# Autodesk Inventor assembly: SMC MSQ Rotary Pneumatic Rack and Pinion Rotary Table Block
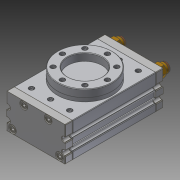
[picture p0: Inventor's stored thumbnail of the model, 180x180]
Saved by Autodesk Inventor 2014 SP1 (Build 180222100, 222)
## iProperties
Created: 2013-12-16
Part Number: SMC MSQ Rotary Pneumatic Rack and Pinion Rotary Table Block
Document SubType Name: Assembly
Designer: Moses
Mass: 511.529 g
Surface Area: 776.899 cm^2
Volume: 450.572 cm^3
Density: 1.13529 g/cm^3
Author: Moses
## Documents named in this file (7)
- C:\Users\Moses\Documents\Inventor\Sally Rebuild\Rebuild Sally\SMC MSQ Rotary Pneumatic Rack and Pinion Rotary Table Block.iam
- C:\Users\Moses\Documents\Inventor\Sally Rebuild\Rebuild Sally\Rotary Pneumatic Cylinder Body.ipt
- C:\Users\Moses\Documents\Inventor\Sally Rebuild\Rebuild Sally\Rotary Pneumatic Cylinder Front End.ipt
- C:\Users\Moses\Documents\Inventor\Sally Rebuild\Rebuild Sally\Rotary Pneumatic Cylinder Back End.ipt
- C:\Users\Moses\Documents\Inventor\Sally Rebuild\Rebuild Sally\Rotary Pneumatic Cylinder Axis.ipt
- C:\Users\Moses\Documents\Inventor\Sally Rebuild\Rebuild Sally\Pneumatics\Pneumatics_SMC_KQ2H07-35S.ipt
- C:\Users\Moses\Documents\Inventor\Sally Rebuild\Rebuild Sally\10-32x0625_shcs.ipt
## Components (14 placed, 6 different names)
1. Rotary Pneumatic Cylinder Body:1 — Mate:1, Flush:1, Flush:2, Mate:2, Flush:3, Flush:4, Insert:1
2. Rotary Pneumatic Cylinder Front End:1 — Mate:1, Flush:1, Flush:2, Insert:8, Insert:9, Insert:10, Insert:11
3. Rotary Pneumatic Cylinder Back End:1 — Mate:2, Flush:3, Flush:4, Insert:2, Insert:3, Insert:4, Insert:5, Insert:6, Insert:7
4. Rotary Pneumatic Cylinder Axis:1 — Insert:1
5. Pneumatics_SMC_KQ2H07-35S:1 — Insert:2
6. Pneumatics_SMC_KQ2H07-35S:2 — Insert:3
7. 10-32x0625_shcs:1 — Insert:4
8. 10-32x0625_shcs:2 — Insert:5
9. 10-32x0625_shcs:3 — Insert:6
10. 10-32x0625_shcs:4 — Insert:7
11. 10-32x0625_shcs:5 — Insert:8
12. 10-32x0625_shcs:6 — Insert:9
13. 10-32x0625_shcs:7 — Insert:10
14. 10-32x0625_shcs:8 — Insert:11
## Relationships (17: Insert 11, Flush 4, Mate 2)
- Mate:1: Rotary Pneumatic Cylinder Body:1 ↔ Rotary Pneumatic Cylinder Front End:1
- Flush:1: Rotary Pneumatic Cylinder Body:1 ↔ Rotary Pneumatic Cylinder Front End:1
- Flush:2: Rotary Pneumatic Cylinder Body:1 ↔ Rotary Pneumatic Cylinder Front End:1
- Mate:2: Rotary Pneumatic Cylinder Body:1 ↔ Rotary Pneumatic Cylinder Back End:1
- Flush:3: Rotary Pneumatic Cylinder Body:1 ↔ Rotary Pneumatic Cylinder Back End:1
- Flush:4: Rotary Pneumatic Cylinder Body:1 ↔ Rotary Pneumatic Cylinder Back End:1
- Insert:1: Rotary Pneumatic Cylinder Body:1 ↔ Rotary Pneumatic Cylinder Axis:1
- Insert:2 (1.27 mm): Rotary Pneumatic Cylinder Back End:1 ↔ Pneumatics_SMC_KQ2H07-35S:1
- Insert:3 (1.27 mm): Rotary Pneumatic Cylinder Back End:1 ↔ Pneumatics_SMC_KQ2H07-35S:2
- Insert:4: Rotary Pneumatic Cylinder Back End:1 ↔ 10-32x0625_shcs:1
- Insert:5: Rotary Pneumatic Cylinder Back End:1 ↔ 10-32x0625_shcs:2
- Insert:6: Rotary Pneumatic Cylinder Back End:1 ↔ 10-32x0625_shcs:3
- Insert:7: Rotary Pneumatic Cylinder Back End:1 ↔ 10-32x0625_shcs:4
- Insert:8: Rotary Pneumatic Cylinder Front End:1 ↔ 10-32x0625_shcs:5
- Insert:9: Rotary Pneumatic Cylinder Front End:1 ↔ 10-32x0625_shcs:6
- Insert:10: Rotary Pneumatic Cylinder Front End:1 ↔ 10-32x0625_shcs:7
- Insert:11: Rotary Pneumatic Cylinder Front End:1 ↔ 10-32x0625_shcs:8
